# Autodesk Inventor assembly: AssemblyFinal01
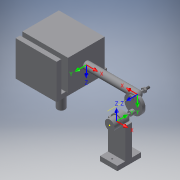
[picture p0: Inventor's stored thumbnail of the model, 180x180]
Saved by Autodesk Inventor 2019 (Build 230136000, 136)
## iProperties
Created: 2019-10-20
Part Number: AssemblyFinal01
Document SubType Name: Assembly
Designer: sudhanva
Author: sudhanva
## Documents named in this file (3)
- E:\Engineering softwares\3D Design\AssemblyFinal01.iam
- E:\Engineering softwares\3D Design\Mechanism Final.iam
- E:\Engineering softwares\3D Design\2.ipt
## Components (2 placed, 2 different names)
1. Mechanism Final:1 [sub-assembly] — Rigid:1
2. 2:1 — Rigid:1
## Relationships (1: WeldJoint 1)
- Rigid:1 [WeldJoint]: Mechanism Final:1 ↔ 2:1
